# Autodesk Inventor assembly: complete-gimbal
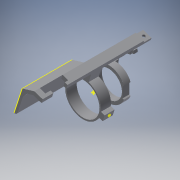
[picture p0: Inventor's stored thumbnail of the model, 180x180]
Saved by Autodesk Inventor 2017 (Build 210142000, 142)
## iProperties
Part Number: complete-gimbal
Material: 常规
Document SubType Name: Assembly
Designer: Lenovo
Author: Lenovo
## Documents named in this file (3)
- C:\Users\Lenovo\Documents\complete-gimbal.iam
- C:\Users\Lenovo\Documents\X-axis-gimbal-part.ipt
- C:\Users\Lenovo\Documents\Y-axis-gimbal-part-scaled.ipt
## Components (2 placed, 2 different names)
1. X-axis-gimbal-part:1 — Mate:1, Flush:1
2. Y-axis-gimbal-part-scaled:1 — Mate:1, Flush:1
## Relationships (2: Mate 1, Flush 1)
- Mate:1: X-axis-gimbal-part:1 ↔ Y-axis-gimbal-part-scaled:1
- Flush:1 (-50 mm): X-axis-gimbal-part:1 ↔ Y-axis-gimbal-part-scaled:1
